# Autodesk Inventor assembly: Claw2017-18
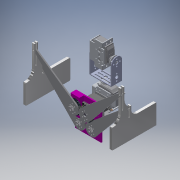
[picture p0: Inventor's stored thumbnail of the model, 180x180]
Saved by Autodesk Inventor 2017 (Build 210142000, 142)
## iProperties
Created: 2017-09-28
Part Number: Claw2017-18
Document SubType Name: Assembly
Designer: User
Author: User
## Documents named in this file (11)
- C:\Robotics\CAD\2017-18_CAD\Claw2017-18 - backup.iam
- C:\Robotics\CAD\2017-18_CAD\ClawServoHolder.ipt
- C:\Robotics\CAD\COTSParts\Tetrix\Tetrix servo 180.ipt
- C:\Robotics\CAD\COTSParts\Tetrix\Tetrix Gear 40T.ipt
- C:\Robotics\CAD\2017-18_CAD\ClawLinkage.ipt
- C:\Robotics\CAD\2017-18_CAD\2BarClawPaddle.ipt
- C:\Robotics\CAD\COTSParts\Vex\91259A576_ALLOY STEEL SHOULDER SCREW.ipt
- C:\Robotics\CAD\COTSParts\Tetrix\Tetrix bracket - single servo.ipt
- C:\Robotics\CAD\2017-18_CAD\TheClaw.iam
- C:\Robotics\CAD\2017-18_CAD\97345A201_TYPE 316 STAINLESS STEEL SHOULDER SCREW.ipt
- C:\Robotics\CAD\2017-18_CAD\2BarClawPaddle2.0.ipt
## Components (17 placed, 10 different names)
1. ClawServoHolder:1 — Mate:5, Mate:6, Mate:7, Mate:11, Mate:12, Mate:43, Mate:44, Mate:55, Mate:58, Mate:63, Mate:64
2. Tetrix servo 180:1 — Mate:5, Mate:6, Mate:7, Mate:9, Mate:10, Mate:56, Mate:57
3. Tetrix Gear 40T:1 — Mate:9, Mate:10, Flush:5, Mate:19, Mate:20, Mate:21
4. Tetrix Gear 40T:2 — Mate:11, Mate:12, Flush:5, Mate:22, Mate:23, Mate:24
5. ClawLinkage:1 — Mate:19, Mate:20, Mate:21, Mate:59, Mate:60, Mate:66
6. ClawLinkage:2 — Mate:22, Mate:23, Mate:24, Mate:42, Mate:69
7. 2BarClawPaddle:2 — Mate:42
8. 91259A576_ALLOY STEEL SHOULDER SCREW:1 — Mate:43, Mate:44
9. ClawLinkage:3 — Mate:61, Mate:62, Insert:7
10. ClawLinkage:4 — Mate:58, Insert:6, Mate:67, Mate:68
11. Tetrix bracket - single servo:1 — Mate:55, Mate:56, Insert:4, Insert:5, Mate:57
12. TheClaw:1 [sub-assembly] — Insert:4, Insert:5
13. 2BarClawPaddle:3 — Mate:59, Mate:60, Mate:61, Mate:62
14. 97345A201_TYPE 316 STAINLESS STEEL SHOULDER SCREW:1 — Mate:64, Insert:6
15. 97345A201_TYPE 316 STAINLESS STEEL SHOULDER SCREW:2 — Mate:63, Insert:7
16. 2BarClawPaddle2.0:1 — Mate:66
17. 2BarClawPaddle2.0:2 — Mate:67, Mate:68, Mate:69
## Relationships (35: Mate 30, Insert 4, Flush 1)
- Mate:5: ClawServoHolder:1 ↔ Tetrix servo 180:1
- Mate:6: ClawServoHolder:1 ↔ Tetrix servo 180:1
- Mate:7: ClawServoHolder:1 ↔ Tetrix servo 180:1
- Mate:9: Tetrix servo 180:1 ↔ Tetrix Gear 40T:1
- Mate:10: Tetrix servo 180:1 ↔ Tetrix Gear 40T:1
- Mate:11: ClawServoHolder:1 ↔ Tetrix Gear 40T:2
- Mate:12: ClawServoHolder:1 ↔ Tetrix Gear 40T:2
- Flush:5: Tetrix Gear 40T:1 ↔ Tetrix Gear 40T:2
- Mate:19: Tetrix Gear 40T:1 ↔ ClawLinkage:1
- Mate:20: Tetrix Gear 40T:1 ↔ ClawLinkage:1
- Mate:21: Tetrix Gear 40T:1 ↔ ClawLinkage:1
- Mate:22: Tetrix Gear 40T:2 ↔ ClawLinkage:2
- Mate:23: Tetrix Gear 40T:2 ↔ ClawLinkage:2
- Mate:24: Tetrix Gear 40T:2 ↔ ClawLinkage:2
- Mate:42: ClawLinkage:2 ↔ 2BarClawPaddle:2
- Mate:43: ClawServoHolder:1 ↔ 91259A576_ALLOY STEEL SHOULDER SCREW:1
- Mate:44: ClawServoHolder:1 ↔ 91259A576_ALLOY STEEL SHOULDER SCREW:1
- Mate:55 (2.54 mm): ClawServoHolder:1 ↔ Tetrix bracket - single servo:1
- Mate:56: Tetrix servo 180:1 ↔ Tetrix bracket - single servo:1
- Insert:4: Tetrix bracket - single servo:1 ↔ TheClaw:1
- Insert:5: Tetrix bracket - single servo:1 ↔ TheClaw:1
- Mate:57: Tetrix servo 180:1 ↔ Tetrix bracket - single servo:1
- Mate:58: ClawServoHolder:1 ↔ ClawLinkage:4
- Mate:59: ClawLinkage:1 ↔ 2BarClawPaddle:3
- Mate:60: ClawLinkage:1 ↔ 2BarClawPaddle:3
- Mate:61: ClawLinkage:3 ↔ 2BarClawPaddle:3
- Mate:62: ClawLinkage:3 ↔ 2BarClawPaddle:3
- Mate:63: ClawServoHolder:1 ↔ 97345A201_TYPE 316 STAINLESS STEEL SHOULDER SCREW:2
- Mate:64: ClawServoHolder:1 ↔ 97345A201_TYPE 316 STAINLESS STEEL SHOULDER SCREW:1
- Insert:6: ClawLinkage:4 ↔ 97345A201_TYPE 316 STAINLESS STEEL SHOULDER SCREW:1
- Insert:7: ClawLinkage:3 ↔ 97345A201_TYPE 316 STAINLESS STEEL SHOULDER SCREW:2
- Mate:66: ClawLinkage:1 ↔ 2BarClawPaddle2.0:1
- Mate:67: ClawLinkage:4 ↔ 2BarClawPaddle2.0:2
- Mate:68: ClawLinkage:4 ↔ 2BarClawPaddle2.0:2
- Mate:69: ClawLinkage:2 ↔ 2BarClawPaddle2.0:2
